# Autodesk Inventor assembly: EnsamblajeGruaSTD
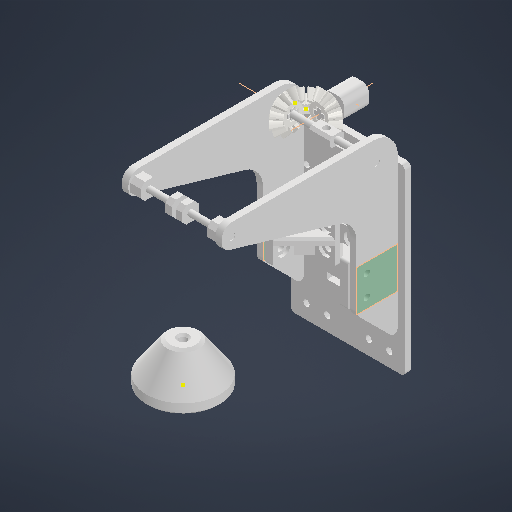
[picture p0: Inventor's stored thumbnail of the model, 512x512]
Saved by Autodesk Inventor 2026.2 (Build 302298010, 298A)
## iProperties
Created: 2026-04-22
Part Number: EnsamblajeGruaSTD
Document SubType Name: Assembly
Designer: Jose Carlos
Author: Jose Carlos
## Documents named in this file (13)
- D:\TEC\Cursos\TFG\Inventor\PiezasSTD\EnsambleGruaSTD\EnsamblajeGruaSTD.iam
- D:\TEC\Cursos\TFG\Inventor\PiezasSTD\PlacaFrontalSTD.ipt
- D:\TEC\Cursos\TFG\Inventor\PiezasSTD\T.ipt
- D:\TEC\Cursos\TFG\Inventor\PiezasSTD\PlacaBaseGarraPotenciaSTD.ipt
- D:\TEC\Cursos\TFG\Inventor\PiezasSTD\SoporteEjes.ipt
- D:\TEC\Cursos\TFG\Inventor\PiezasSTD\EjeCilintroSuperiorGarra.ipt
- D:\TEC\Cursos\TFG\Inventor\PiezasSTD\EnsambleGarraSTD\Design Accelerator\Engranaje biselado11.ipt
- D:\TEC\Cursos\TFG\Inventor\PiezasSTD\EnsambleGruaSTD\EjeCortoGrua.ipt
- D:\TEC\Cursos\TFG\Inventor\PiezasSTD\Acoplador.ipt
- D:\TEC\Cursos\TFG\Inventor\PiezasSTD\EnsambleGruaSTD\ParedLateralGrua1.ipt
- D:\TEC\Cursos\TFG\Inventor\PiezasSTD\EnsambleGruaSTD\EjeEngraneGrua.ipt
- D:\TEC\Cursos\TFG\Inventor\PiezasSTD\EnsambleGruaSTD\EjeFrontalGrúa.ipt
- D:\TEC\Cursos\TFG\Inventor\PiezasSTD\EnsambleGruaSTD\PesaGrua.ipt
## Components (15 placed, 12 different names)
1. T:1 — Coincidencia:1, Ángulo:1, Nivelación:1, Coincidencia:2, Nivelación:17, Nivelación:18
2. T:2 — Ángulo:2, Coincidencia:3, Nivelación:2, Coincidencia:4, Ángulo:5, Coincidencia:15, Coincidencia:16
3. PlacaFrontalSTD:1 — Coincidencia:1, Ángulo:1, Nivelación:1, Coincidencia:2, Ángulo:2, Coincidencia:3, Nivelación:2, Coincidencia:4, Nivelación:6, Nivelación:7, Coincidencia:5, Coincidencia:10, Ángulo:3, Coincidencia:11, Nivelación:15, Nivelación:16, Ángulo:4, Coincidencia:14
4. PlacaBaseGarraPotenciaSTD:1 — Nivelación:6, Nivelación:7, Coincidencia:5, Coincidencia:6, Coincidencia:7
5. SoporteEjes:1 — Coincidencia:6, Coincidencia:7, Nivelación:8, Coincidencia:8
6. EjeCilintroSuperiorGarra:1 — Nivelación:8, Coincidencia:8, Coincidencia:9, Nivelación:9, Nivelación:10, Nivelación:11
7. Engranaje biselado1:1 — Coincidencia:9, Coincidencia:10, Coincidencia:12, Coincidencia:13
8. Engranaje biselado1:2 — Ángulo:3, Coincidencia:12, Ángulo:5
9. EjeCortoGrua:1 — Nivelación:9, Nivelación:10, Nivelación:11, Nivelación:12, Nivelación:13, Nivelación:14, Nivelación:27
10. Acoplador:1 — Nivelación:12, Nivelación:13, Nivelación:14, Coincidencia:13, Ángulo:4, Nivelación:27
11. ParedLateralGrua1:1 — Nivelación:17, Nivelación:18, Nivelación:19, Nivelación:20, Nivelación:22, Nivelación:23, Nivelación:24, Nivelación:26
12. ParedLateralGrua1:2 — Coincidencia:14, Coincidencia:15, Coincidencia:16, Nivelación:21, Nivelación:25
13. EjeEngraneGrua:1 — Nivelación:19, Nivelación:20, Nivelación:21, Nivelación:22
14. EjeFrontalGrúa:1 — Nivelación:23, Nivelación:24, Nivelación:25, Nivelación:26
15. PesaGrua:1
## Relationships (45: Flush 24, Mate 16, Angle 5)
- Coincidencia:1 [Mate]: T:1 ↔ PlacaFrontalSTD:1
- Ángulo:1 [Angle] (180 deg): T:1 ↔ PlacaFrontalSTD:1
- Nivelación:1 [Flush] (1 mm): T:1 ↔ PlacaFrontalSTD:1
- Coincidencia:2 [Mate]: T:1 ↔ PlacaFrontalSTD:1
- Ángulo:2 [Angle] (0 deg): T:2 ↔ PlacaFrontalSTD:1
- Coincidencia:3 [Mate]: T:2 ↔ PlacaFrontalSTD:1
- Nivelación:2 [Flush]: T:2 ↔ PlacaFrontalSTD:1
- Coincidencia:4 [Mate] (1 mm): T:2 ↔ PlacaFrontalSTD:1
- Nivelación:6 [Flush]: PlacaFrontalSTD:1 ↔ PlacaBaseGarraPotenciaSTD:1
- Nivelación:7 [Flush]: PlacaFrontalSTD:1 ↔ PlacaBaseGarraPotenciaSTD:1
- Coincidencia:5 [Mate]: PlacaFrontalSTD:1 ↔ PlacaBaseGarraPotenciaSTD:1
- Coincidencia:6 [Mate]: PlacaBaseGarraPotenciaSTD:1 ↔ SoporteEjes:1
- Coincidencia:7 [Mate]: PlacaBaseGarraPotenciaSTD:1 ↔ SoporteEjes:1
- Nivelación:8 [Flush]: SoporteEjes:1 ↔ EjeCilintroSuperiorGarra:1
- Coincidencia:8 [Mate]: SoporteEjes:1 ↔ EjeCilintroSuperiorGarra:1
- Coincidencia:9 [Mate]: EjeCilintroSuperiorGarra:1 ↔ Engranaje biselado1:1
- Coincidencia:10 [Mate]: PlacaFrontalSTD:1 ↔ Engranaje biselado1:1
- Nivelación:9 [Flush]: EjeCilintroSuperiorGarra:1 ↔ EjeCortoGrua:1
- Nivelación:10 [Flush]: EjeCilintroSuperiorGarra:1 ↔ EjeCortoGrua:1
- Nivelación:11 [Flush]: EjeCilintroSuperiorGarra:1 ↔ EjeCortoGrua:1
- Nivelación:12 [Flush]: EjeCortoGrua:1 ↔ Acoplador:1
- Nivelación:13 [Flush]: EjeCortoGrua:1 ↔ Acoplador:1
- Nivelación:14 [Flush]: EjeCortoGrua:1 ↔ Acoplador:1
- Ángulo:3 [Angle] (0 deg): PlacaFrontalSTD:1 ↔ Engranaje biselado1:2
- Coincidencia:11 [Mate]: PlacaFrontalSTD:1
- Nivelación:15 [Flush]: PlacaFrontalSTD:1
- Nivelación:16 [Flush]: PlacaFrontalSTD:1
- Coincidencia:12 [Mate]: Engranaje biselado1:1 ↔ Engranaje biselado1:2
- Coincidencia:13 [Mate]: Engranaje biselado1:1 ↔ Acoplador:1
- Ángulo:4 [Angle] (0 deg): PlacaFrontalSTD:1 ↔ Acoplador:1
- Ángulo:5 [Angle] (0 deg): T:2 ↔ Engranaje biselado1:2
- Nivelación:17 [Flush]: T:1 ↔ ParedLateralGrua1:1
- Nivelación:18 [Flush]: T:1 ↔ ParedLateralGrua1:1
- Coincidencia:14 [Mate]: PlacaFrontalSTD:1 ↔ ParedLateralGrua1:2
- Coincidencia:15 [Mate]: T:2 ↔ ParedLateralGrua1:2
- Coincidencia:16 [Mate]: T:2 ↔ ParedLateralGrua1:2
- Nivelación:19 [Flush]: ParedLateralGrua1:1 ↔ EjeEngraneGrua:1
- Nivelación:20 [Flush]: ParedLateralGrua1:1 ↔ EjeEngraneGrua:1
- Nivelación:21 [Flush]: ParedLateralGrua1:2 ↔ EjeEngraneGrua:1
- Nivelación:22 [Flush]: ParedLateralGrua1:1 ↔ EjeEngraneGrua:1
- Nivelación:23 [Flush]: ParedLateralGrua1:1 ↔ EjeFrontalGrúa:1
- Nivelación:24 [Flush]: ParedLateralGrua1:1 ↔ EjeFrontalGrúa:1
- Nivelación:25 [Flush]: ParedLateralGrua1:2 ↔ EjeFrontalGrúa:1
- Nivelación:26 [Flush]: ParedLateralGrua1:1 ↔ EjeFrontalGrúa:1
- Nivelación:27 [Flush]: EjeCortoGrua:1 ↔ Acoplador:1
